# Autodesk Inventor assembly: untitled.brd
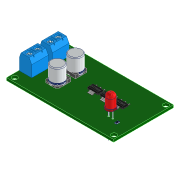
[picture p0: Inventor's stored thumbnail of the model, 180x180]
Saved by Autodesk Inventor 2022 (Build 260153000, 153)
## iProperties
Created: 2023-03-06
Part Number: untitled.brd
Document SubType Name: Assembly
Designer: Иван Петров
Author: Иван Петров
## Documents named in this file (8)
- C:\Users\Ivan Petrov\Documents\GitHub\OmniBot\design\000.008 - Бортовой источник питания 3V3 СБ.iam
- C:\Users\Ivan Petrov\Documents\GitHub\OmniBot\design\000.008.001 - Плата печатная.ipt
- C:\Users\Ivan Petrov\Documents\GitHub\OmniBot\design\standart_components\Capacitors smd\05_NICHICON_8X10_NEWARK_58R3566_ENSAMBLE.ipt
- C:\Users\Ivan Petrov\Documents\GitHub\OmniBot\design\standart_components\Terminal Block 2P.ipt
- C:\Users\Ivan Petrov\Documents\GitHub\OmniBot\design\standart_components\LED-Red.ipt
- C:\Users\Ivan Petrov\Documents\GitHub\OmniBot\design\standart_components\smd resistors\0R.iam
- C:\Users\Ivan Petrov\Documents\GitHub\OmniBot\design\standart_components\AMS1117.ipt
- C:\Users\Ivan Petrov\Documents\GitHub\OmniBot\design\000.001.010 - Стойка шестигранная М3 15 мм.ipt
## Components (14 placed, 11 different names)
1. 000.008.001 - Плата печатная — Угол:1, Угол:2, Совмещение:5, Совмещение:6, Совмещение:7, Совмещение:8, Совмещение:9, Совмещение:10, Совмещение:11, Совмещение:12, Совмещение:13, Совмещение:14, Совмещение:15, Угол:3, Совмещение:17, Совмещение:18, Совмещение:19, Совмещение:20, Совмещение:21, Совмещение:22, Совмещение:23, Совмещение:24
2. C9_2 — Совмещение:13, Совмещение:16, Угол:4, Заподлицо:1
3. C10_3 — Совмещение:12, Совмещение:14, Совмещение:15, Совмещение:16, Угол:3, Угол:4, Заподлицо:1
4. J1_5 — Угол:1, Совмещение:5, Совмещение:6
5. J2_7 — Угол:2, Совмещение:7, Совмещение:8
6. LED2_9 — Совмещение:9, Совмещение:10, Совмещение:11
7. R6_11 [sub-assembly]
8. U1_13
9. U2_15
10. U3_17
11. 000.001.010 - Стойка шестигранная М3 15 мм:1 — Совмещение:18, Совмещение:21
12. 000.001.010 - Стойка шестигранная М3 15 мм:2 — Совмещение:17, Совмещение:22
13. 000.001.010 - Стойка шестигранная М3 15 мм:3 — Совмещение:19, Совмещение:23
14. 000.001.010 - Стойка шестигранная М3 15 мм:4 — Совмещение:20, Совмещение:24
## Relationships (25: Mate 20, Angle 4, Flush 1)
- Угол:1 [Angle] (0 deg): 000.008.001 - Плата печатная ↔ J1_5
- Угол:2 [Angle] (0 deg): 000.008.001 - Плата печатная ↔ J2_7
- Совмещение:5 [Mate]: 000.008.001 - Плата печатная ↔ J1_5
- Совмещение:6 [Mate]: 000.008.001 - Плата печатная ↔ J1_5
- Совмещение:7 [Mate]: 000.008.001 - Плата печатная ↔ J2_7
- Совмещение:8 [Mate]: 000.008.001 - Плата печатная ↔ J2_7
- Совмещение:9 [Mate]: 000.008.001 - Плата печатная ↔ LED2_9
- Совмещение:10 [Mate]: 000.008.001 - Плата печатная ↔ LED2_9
- Совмещение:11 [Mate] (5 mm): 000.008.001 - Плата печатная ↔ LED2_9
- Совмещение:12 [Mate]: 000.008.001 - Плата печатная ↔ C10_3
- Совмещение:13 [Mate]: 000.008.001 - Плата печатная ↔ C9_2
- Совмещение:14 [Mate] (-13.461 mm): 000.008.001 - Плата печатная ↔ C10_3
- Совмещение:15 [Mate] (-17.729 mm): 000.008.001 - Плата печатная ↔ C10_3
- Совмещение:16 [Mate] (11.179 mm): C9_2 ↔ C10_3
- Угол:3 [Angle] (0 deg): 000.008.001 - Плата печатная ↔ C10_3
- Угол:4 [Angle] (0 deg): C9_2 ↔ C10_3
- Заподлицо:1 [Flush]: C9_2 ↔ C10_3
- Совмещение:17 [Mate]: 000.008.001 - Плата печатная ↔ 000.001.010 - Стойка шестигранная М3 15 мм:2
- Совмещение:18 [Mate]: 000.008.001 - Плата печатная ↔ 000.001.010 - Стойка шестигранная М3 15 мм:1
- Совмещение:19 [Mate]: 000.008.001 - Плата печатная ↔ 000.001.010 - Стойка шестигранная М3 15 мм:3
- Совмещение:20 [Mate]: 000.008.001 - Плата печатная ↔ 000.001.010 - Стойка шестигранная М3 15 мм:4
- Совмещение:21 [Mate]: 000.008.001 - Плата печатная ↔ 000.001.010 - Стойка шестигранная М3 15 мм:1
- Совмещение:22 [Mate]: 000.008.001 - Плата печатная ↔ 000.001.010 - Стойка шестигранная М3 15 мм:2
- Совмещение:23 [Mate]: 000.008.001 - Плата печатная ↔ 000.001.010 - Стойка шестигранная М3 15 мм:3
- Совмещение:24 [Mate]: 000.008.001 - Плата печатная ↔ 000.001.010 - Стойка шестигранная М3 15 мм:4
